# Autodesk Inventor assembly: Case-ASMB
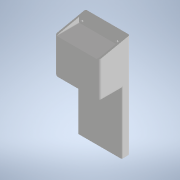
[picture p0: Inventor's stored thumbnail of the model, 180x180]
Saved by Autodesk Inventor 2022 (Build 260153000, 153)
## iProperties
Created: 2023-12-02
Part Number: Case-ASMB
Document SubType Name: Assembly
Designer: Egor
Author: Egor
## Documents named in this file (5)
- C:\Study\Artemiev\case\Case-ASMB.iam
- C:\Study\Artemiev\case\Top.ipt
- C:\Study\Artemiev\case\pcb\PCB1.iam
- C:\Study\Artemiev\case\Case.ipt
- C:\Study\Artemiev\case\Temp_Module.ipt
## Components (4 placed, 4 different names)
1. Top:1 — С поворотом:1, С поворотом:2
2. PCB1:1 [sub-assembly] — С поворотом:1
3. Case:1 — С поворотом:2
4. Temp_Module:1
## Relationships (2: RevoluteJoint 2)
- С поворотом:1 [RevoluteJoint]: Top:1 ↔ PCB1:1
- С поворотом:2 [RevoluteJoint]: Top:1 ↔ Case:1
